# Autodesk Inventor assembly: Nylon-Nylon-Alu
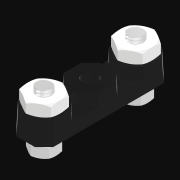
[picture p0: Inventor's stored thumbnail of the model, 180x180]
Saved by Autodesk Inventor 2021 (Build 250183000, 183)
## iProperties
Created: 2020-12-24
Part Number: Nylon-Nylon-Alu
Document SubType Name: Assembly
Designer: yuany
Author: yuany
## Documents named in this file (5)
- E:\VEX Cad\Assembly\Winter Rebuild\Parts with Screws\Nylon-Nylon-Alu.iam
- E:\VEX Cad\Library 1.2\Motion\Bearing Flat.ipt
- E:\VEX Cad\Library 1.2\Structure\Hardware\Nut Nylon - White.ipt
- E:\VEX Cad\Library 1.2\Structure\Hardware\nylon\Nylon .5.ipt
- E:\VEX Cad\Library 1.2\Structure\Hardware\nylon.ipt
## Components (5 placed, 3 different names)
1. Bearing Flat:1 — Insert:1, Insert:2, Mate:1, Mate:2
2. Nut Nylon - White:1 — Insert:1, Mate:3
3. Nut Nylon - White:2 — Insert:2, Mate:4
4. Nylon .5:1 — Mate:1, Mate:4
5. Nylon .5:2 — Mate:2, Mate:3
## Relationships (6: Mate 4, Insert 2)
- Insert:1: Bearing Flat:1 ↔ Nut Nylon - White:1
- Insert:2: Bearing Flat:1 ↔ Nut Nylon - White:2
- Mate:1 (1.6002 mm): Bearing Flat:1 ↔ Nylon .5:1
- Mate:2 (1.6002 mm): Bearing Flat:1 ↔ Nylon .5:2
- Mate:3: Nut Nylon - White:1 ↔ Nylon .5:2
- Mate:4: Nut Nylon - White:2 ↔ Nylon .5:1
